# Autodesk Inventor assembly: Lever
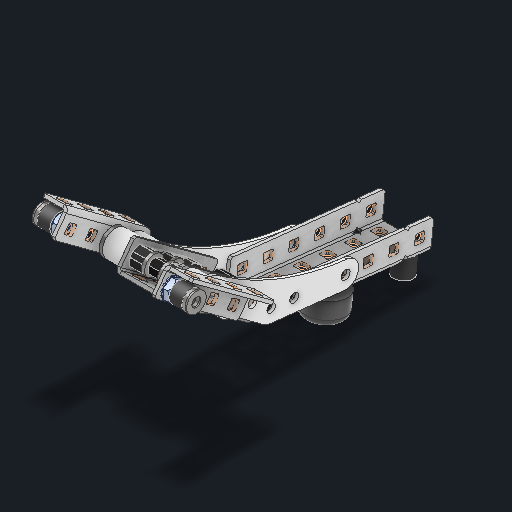
[picture p0: Inventor's stored thumbnail of the model, 512x512]
Saved by Autodesk Inventor 2025.1 (Build 291241000, 241)
## iProperties
Created: 2024-10-22
Part Number: Lever
Document SubType Name: Assembly
Designer: averey
Author: averey
## Documents named in this file (23)
- C:\Users\avere\VEX\High Stakes\CAD\V2\Clamp\Lever.iam
- C:\Users\avere\VEX\High Stakes\CAD\ROBOPROS-CAD-Inventor\Structure\C Channel\Aluminum 1x2x1\Alu C 1x2x1x5.ipt
- C:\Users\avere\VEX\High Stakes\CAD\V2\Clamp\Custom Parts\60 Degree Gusset.ipt
- C:\Users\avere\VEX\High Stakes\CAD\ROBOPROS-CAD-Inventor\Structure\Standoff\Standoff 1.00.ipt
- C:\Users\avere\VEX\High Stakes\CAD\ROBOPROS-CAD-Inventor\Structure\C Channel\Aluminum 1x2x1\Alu C 1x2x1x4.ipt
- C:\Users\avere\VEX\High Stakes\CAD\ROBOPROS-CAD-Inventor\Structure\C Channel\Aluminum 1x2x1\Alu C 1x2x1x6.ipt
- C:\Users\avere\VEX\High Stakes\CAD\ROBOPROS-CAD-Inventor\Structure\Hardware\Rubber Bumper Smooth.ipt
- C:\Users\avere\VEX\High Stakes\CAD\ROBOPROS-CAD-Inventor\Structure\C Channel\Aluminum 1x2x1\Alu C 1x2x1x7.ipt
- C:\Users\avere\VEX\High Stakes\CAD\ROBOPROS-CAD-Inventor\Motion\Spacers\Spacer Nylon .375 OD\NSpacer .375 OD x .375.ipt
- C:\Users\avere\VEX\High Stakes\CAD\ROBOPROS-CAD-Inventor\Motion\Spacers\Spacer Nylon .375 OD.ipt
- C:\Users\avere\VEX\High Stakes\CAD\ROBOPROS-CAD-Inventor\Motion\Spacers\Spacer Nylon .500 OD.ipt
- C:\Users\avere\VEX\High Stakes\CAD\ROBOPROS-CAD-Inventor\Motion\Spacers\Spacer Nylon .500 OD\NSpacer White .500 OD x .375.ipt
- C:\Users\avere\VEX\High Stakes\CAD\ROBOPROS-CAD-Inventor\Motion\Spacers\Washer Steel\SWasher .500 OD x .062500\SWasher .500 OD x .062500.ipt
- C:\Users\avere\VEX\High Stakes\CAD\ROBOPROS-CAD-Inventor\Motion\Spacers\Washer Steel\SWasher .500 OD x .062500.ipt
- C:\Users\avere\VEX\High Stakes\CAD\ROBOPROS-CAD-Inventor\Motion\Shaft LS\Bearing Flat Low Profile.ipt
- C:\Users\avere\VEX\High Stakes\CAD\ROBOPROS-CAD-Inventor\Motion\Spacers\Washer Steel\SWasher .375 OD x .062500.ipt
- C:\Users\avere\VEX\High Stakes\CAD\ROBOPROS-CAD-Inventor\Motion\Spacers\Washer Steel.ipt
- C:\Users\avere\VEX\High Stakes\CAD\ROBOPROS-CAD-Inventor\Structure\Standoff\Standoff .25.ipt
- C:\Users\avere\VEX\High Stakes\CAD\ROBOPROS-CAD-Inventor\Structure\Standoff.ipt
- C:\Users\avere\VEX\High Stakes\CAD\ROBOPROS-CAD-Inventor\Structure\Angle\Aluminum 1x1\Alu Angle 1x1x4.ipt
- C:\Users\avere\VEX\High Stakes\CAD\ROBOPROS-CAD-Inventor\Structure\Hardware\Nut Keps.ipt
- C:\Users\avere\VEX\High Stakes\CAD\ROBOPROS-CAD-Inventor\Motion\Spacers\Spacer Nylon .375 OD\NSpacer .375 OD x .250.ipt
- C:\Users\avere\VEX\High Stakes\CAD\ROBOPROS-CAD-Inventor\Motion\Spacers\Washer Steel\SWasher .375 OD x .031250.ipt
## Components (35 placed, 17 different names)
1. Alu C 1x2x1x5:2 — Insert:2, Insert:3, Insert:6, Mate:7
2. 60 Degree Gusset:1 — Insert:2, Insert:5, Mate:6, Insert:44, Insert:53, Mate:16
3. 60 Degree Gusset:2 — Insert:3, Insert:4, Insert:41
4. Standoff 1.00:1 — Insert:4
5. Alu C 1x2x1x4:1 — Insert:5, Mate:6, Insert:33, Mate:11, Insert:34, Mate:12, Insert:42, Insert:46
6. Alu C 1x2x1x6:1 — Insert:6, Mate:7
7. Rubber Bumper Smooth:1 — Insert:49
8. Alu C 1x2x1x7:1 — Insert:47, Insert:48, Insert:49, Insert:52, Mate:15
9. Bearing Flat Low Profile:1 — Insert:34, Mate:12, Insert:37, Insert:38
10. Bearing Flat Low Profile:2 — Insert:33, Mate:11, Insert:35, Insert:36
11. SWasher .375 OD x .062500:1 — Insert:35
12. SWasher .375 OD x .062500:2 — Insert:36
13. SWasher .375 OD x .062500:3 — Insert:37, Insert:39
14. SWasher .375 OD x .062500:4 — Insert:38, Insert:40
15. Standoff .25:2 — Insert:40
16. Standoff .25:3 — Insert:39
17. SWasher .500 OD x .062500:3 — Insert:43
18. NSpacer White .500 OD x .375:3 — Insert:41, Insert:50
19. NSpacer White .500 OD x .375:4 — Insert:42, Insert:43, Mate:13
20. NSpacer White .500 OD x .375:5 — Insert:44, Insert:51
21. SWasher .500 OD x .062500:4 — Mate:14
22. NSpacer White .500 OD x .375:6 — Insert:46
23. NSpacer .375 OD x .375:1 — Insert:47
24. NSpacer .375 OD x .375:2 — Insert:48
25. Alu Angle 1x1x4:1 — Insert:51, Mate:14, Insert:54
26. Alu Angle 1x1x4:2 — Insert:50, Mate:13, Insert:55
27. Alu C 1x2x1x6:2 — Insert:52, Mate:15, Insert:53, Mate:16
28. Nut Keps:1 — Insert:54, Insert:58
29. Nut Keps:2 — Insert:55, Insert:61
30. NSpacer .375 OD x .250:3 — Insert:57, Insert:58
31. SWasher .375 OD x .031250:5 — Insert:56
32. SWasher .375 OD x .062500:6 — Insert:56, Insert:57
33. NSpacer .375 OD x .250:4 — Insert:61
34. SWasher .375 OD x .031250:7
35. SWasher .375 OD x .062500:8
## Relationships (42: Insert 34, Mate 8)
- Insert:2: Alu C 1x2x1x5:2 ↔ 60 Degree Gusset:1
- Insert:3: Alu C 1x2x1x5:2 ↔ 60 Degree Gusset:2
- Insert:4: 60 Degree Gusset:2 ↔ Standoff 1.00:1
- Insert:5: 60 Degree Gusset:1 ↔ Alu C 1x2x1x4:1
- Mate:6: 60 Degree Gusset:1 ↔ Alu C 1x2x1x4:1
- Insert:6: Alu C 1x2x1x5:2 ↔ Alu C 1x2x1x6:1
- Mate:7: Alu C 1x2x1x5:2 ↔ Alu C 1x2x1x6:1
- Insert:33: Alu C 1x2x1x4:1 ↔ Bearing Flat Low Profile:2
- Mate:11: Alu C 1x2x1x4:1 ↔ Bearing Flat Low Profile:2
- Insert:34: Alu C 1x2x1x4:1 ↔ Bearing Flat Low Profile:1
- Mate:12: Alu C 1x2x1x4:1 ↔ Bearing Flat Low Profile:1
- Insert:35 (1.27 mm): Bearing Flat Low Profile:2 ↔ SWasher .375 OD x .062500:1
- Insert:36 (1.27 mm): Bearing Flat Low Profile:2 ↔ SWasher .375 OD x .062500:2
- Insert:37 (1.27 mm): Bearing Flat Low Profile:1 ↔ SWasher .375 OD x .062500:3
- Insert:38 (1.27 mm): Bearing Flat Low Profile:1 ↔ SWasher .375 OD x .062500:4
- Insert:39: SWasher .375 OD x .062500:3 ↔ Standoff .25:3
- Insert:40: SWasher .375 OD x .062500:4 ↔ Standoff .25:2
- Insert:41: 60 Degree Gusset:2 ↔ NSpacer White .500 OD x .375:3
- Insert:42: Alu C 1x2x1x4:1 ↔ NSpacer White .500 OD x .375:4
- Insert:43: SWasher .500 OD x .062500:3 ↔ NSpacer White .500 OD x .375:4
- Insert:44: 60 Degree Gusset:1 ↔ NSpacer White .500 OD x .375:5
- [Insert]: SWasher .500 OD x .062500:4 ↔ NSpacer White .500 OD x .375:6
- Insert:46: Alu C 1x2x1x4:1 ↔ NSpacer White .500 OD x .375:6
- Insert:47: Alu C 1x2x1x7:1 ↔ NSpacer .375 OD x .375:1
- Insert:48: Alu C 1x2x1x7:1 ↔ NSpacer .375 OD x .375:2
- Insert:49 (6.35 mm): Rubber Bumper Smooth:1 ↔ Alu C 1x2x1x7:1
- Insert:50: NSpacer White .500 OD x .375:3 ↔ Alu Angle 1x1x4:2
- Mate:13: NSpacer White .500 OD x .375:4 ↔ Alu Angle 1x1x4:2
- Insert:51: NSpacer White .500 OD x .375:5 ↔ Alu Angle 1x1x4:1
- Mate:14: SWasher .500 OD x .062500:4 ↔ Alu Angle 1x1x4:1
- Insert:52: Alu C 1x2x1x7:1 ↔ Alu C 1x2x1x6:2
- Mate:15: Alu C 1x2x1x7:1 ↔ Alu C 1x2x1x6:2
- Insert:53: 60 Degree Gusset:1 ↔ Alu C 1x2x1x6:2
- Mate:16: 60 Degree Gusset:1 ↔ Alu C 1x2x1x6:2
- Insert:54: Alu Angle 1x1x4:1 ↔ Nut Keps:1
- Insert:55: Alu Angle 1x1x4:2 ↔ Nut Keps:2
- Insert:56: SWasher .375 OD x .031250:5 ↔ SWasher .375 OD x .062500:6
- Insert:57: NSpacer .375 OD x .250:3 ↔ SWasher .375 OD x .062500:6
- Insert:58: Nut Keps:1 ↔ NSpacer .375 OD x .250:3
- [Insert]: SWasher .375 OD x .031250:7 ↔ SWasher .375 OD x .062500:8
- [Insert]: NSpacer .375 OD x .250:4 ↔ SWasher .375 OD x .062500:8
- Insert:61: Nut Keps:2 ↔ NSpacer .375 OD x .250:4
## Named parameters: d82_d80 = 0 mm, d104_d101 = 0 mm, d105_d102 = 0 mm
